# Autodesk Inventor assembly: Claw Assembly
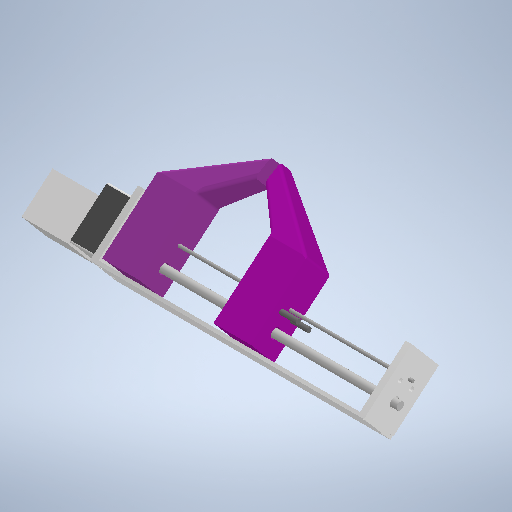
[picture p0: Inventor's stored thumbnail of the model, 512x512]
Saved by Autodesk Inventor 2025.1 (Build 291241020, 241B)
## iProperties
Created: 2025-01-21
Part Number: Claw Assembly
Document SubType Name: Assembly
Designer: Sven
Author: Sven
## Documents named in this file (12)
- C:\Users\aidan\Documents\BehrendURCMechanical\CAD\Arm\Hamburger\BRC Robotic CLaw\Claw Assembly.iam
- C:\Users\aidan\Documents\BehrendURCMechanical\CAD\Arm\Hamburger\BRC Robotic CLaw\Moving Gripper.ipt
- C:\Users\aidan\Documents\BehrendURCMechanical\CAD\Arm\Hamburger\BRC Robotic CLaw\Stationary Gripper.ipt
- C:\Users\aidan\Documents\BehrendURCMechanical\CAD\Arm\Hamburger\BRC Robotic CLaw\Lead Screw.ipt
- C:\Users\aidan\Documents\BehrendURCMechanical\CAD\Arm\Hamburger\BRC Robotic CLaw\#10 2in.ipt
- C:\Users\aidan\Documents\BehrendURCMechanical\CAD\Arm\Hamburger\BRC Robotic CLaw\Support Bar.ipt
- C:\Users\aidan\Documents\BehrendURCMechanical\CAD\Arm\Hamburger\BRC Robotic CLaw\Motor Brace.ipt
- C:\Users\aidan\Documents\BehrendURCMechanical\CAD\Arm\Hamburger\BRC Robotic CLaw\Couple.ipt
- C:\Users\aidan\Documents\BehrendURCMechanical\CAD\Arm\Hamburger\BRC Robotic CLaw\NEMA 17 Completely Correct.ipt
- C:\Users\aidan\Documents\BehrendURCMechanical\CAD\Arm\Hamburger\BRC Robotic CLaw\Bracket(left).ipt
- C:\Users\aidan\Documents\BehrendURCMechanical\CAD\Arm\Hamburger\BRC Robotic CLaw\Bracket(middle).ipt
- C:\Users\aidan\Documents\BehrendURCMechanical\CAD\Arm\Hamburger\BRC Robotic CLaw\Bracket(right).ipt
## Components (12 placed, 11 different names)
1. Moving Gripper:1 — Mate:6, Mate:14, Mate:19, Mate:26, Mate:40
2. Stationary Gripper:1 — Mate:7, Mate:8, Mate:9, Mate:10, Mate:11, Mate:14, Mate:27
3. Lead Screw:1 — Mate:6, Mate:7, Mate:20, Mate:21, Mate:25, Mate:28
4. #10 2in:1 — Mate:8, Mate:9
5. #10 2in:2 — Mate:10, Mate:11
6. Support Bar:1 — Mate:26, Mate:27, Mate:33
7. Motor Brace:1 — Mate:19, Mate:29, Mate:30, Mate:31, Mate:32, Mate:33, Mate:34
8. Couple:1 — Mate:20, Mate:21, Mate:24, Mate:30
9. NEMA 17 Completely Correct:1 — Mate:24, Mate:25, Mate:31, Mate:32
10. Bracket(left):1 — Mate:28, Mate:29, Mate:34, Mate:35, Mate:36, Mate:37, Mate:40
11. Bracket(middle):1 — Mate:35, Mate:36, Mate:37, Mate:38, Mate:39
12. Bracket(right):1 — Mate:38, Mate:39
## Relationships (27: Mate 27)
- Mate:6: Moving Gripper:1 ↔ Lead Screw:1
- Mate:7: Stationary Gripper:1 ↔ Lead Screw:1
- Mate:8: Stationary Gripper:1 ↔ #10 2in:1
- Mate:9: Stationary Gripper:1 ↔ #10 2in:1
- Mate:10: Stationary Gripper:1 ↔ #10 2in:2
- Mate:11: Stationary Gripper:1 ↔ #10 2in:2
- Mate:14: Moving Gripper:1 ↔ Stationary Gripper:1
- Mate:19: Moving Gripper:1 ↔ Motor Brace:1
- Mate:20: Lead Screw:1 ↔ Couple:1
- Mate:21: Lead Screw:1 ↔ Couple:1
- Mate:24: Couple:1 ↔ NEMA 17 Completely Correct:1
- Mate:25: Lead Screw:1 ↔ NEMA 17 Completely Correct:1
- Mate:26: Moving Gripper:1 ↔ Support Bar:1
- Mate:27: Stationary Gripper:1 ↔ Support Bar:1
- Mate:28: Lead Screw:1 ↔ Bracket(left):1
- Mate:29: Motor Brace:1 ↔ Bracket(left):1
- Mate:30: Motor Brace:1 ↔ Couple:1
- Mate:31: Motor Brace:1 ↔ NEMA 17 Completely Correct:1
- Mate:32: Motor Brace:1 ↔ NEMA 17 Completely Correct:1
- Mate:33: Support Bar:1 ↔ Motor Brace:1
- Mate:34: Motor Brace:1 ↔ Bracket(left):1
- Mate:35: Bracket(left):1 ↔ Bracket(middle):1
- Mate:36: Bracket(left):1 ↔ Bracket(middle):1
- Mate:37: Bracket(left):1 ↔ Bracket(middle):1
- Mate:38: Bracket(middle):1 ↔ Bracket(right):1
- Mate:39: Bracket(middle):1 ↔ Bracket(right):1
- Mate:40: Moving Gripper:1 ↔ Bracket(left):1
